# Autodesk Inventor assembly: Carburetor
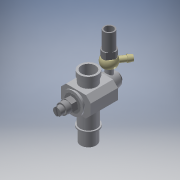
[picture p0: Inventor's stored thumbnail of the model, 180x180]
Saved by Autodesk Inventor 2016 (Build 200138000, 138)
## iProperties
Created: 2012-08-25
Part Number: Carburetor
Document SubType Name: Assembly
Designer: John
Author: John
## Documents named in this file (8)
- C:\File Storage\Autodesk\Inventor 2016 Projects\Ex_Files_Inventor_2016_EssT\Exercise Files\02_Navigating the interface\02_01\Carburetor.iam
- C:\File Storage\Autodesk\Inventor 2016 Projects\Ex_Files_Inventor_2016_EssT\Exercise Files\02_Navigating the interface\02_01\Gas Regulator.ipt
- C:\File Storage\Autodesk\Inventor 2016 Projects\Ex_Files_Inventor_2016_EssT\Exercise Files\02_Navigating the interface\02_01\Mixture Control.ipt
- C:\File Storage\Autodesk\Inventor 2016 Projects\Ex_Files_Inventor_2016_EssT\Exercise Files\02_Navigating the interface\02_01\Air Adjuster.ipt
- C:\File Storage\Autodesk\Inventor 2016 Projects\Ex_Files_Inventor_2016_EssT\Exercise Files\02_Navigating the interface\02_01\Hex Cap.ipt
- C:\File Storage\Autodesk\Inventor 2016 Projects\Ex_Files_Inventor_2016_EssT\Exercise Files\02_Navigating the interface\02_01\Fuel Intake.ipt
- C:\File Storage\Autodesk\Inventor 2016 Projects\Ex_Files_Inventor_2016_EssT\Exercise Files\02_Navigating the interface\02_01\Fuel Adjuster.ipt
- C:\File Storage\Autodesk\Inventor 2016 Projects\Ex_Files_Inventor_2016_EssT\Exercise Files\02_Navigating the interface\02_01\Carburetor Housing_v3.ipt
## Components (7 placed, 7 different names)
1. Carburetor Housing_v3:2 — Mate:6, Mate:7, Mate:10, Flush:1, Flush:2
2. Gas Regulator:1 — Mate:6, Flush:1
3. Mixture Control:1 — Flush:2
4. Air Adjuster:1
5. Hex Cap:1
6. Fuel Intake:1 — Mate:8, Mate:9, Mate:10
7. Fuel Adjuster:1 — Mate:7, Mate:8, Mate:9
## Relationships (12: Mate 10, Flush 2)
- [Mate]: Gas Regulator:1 ↔ Mixture Control:1
- [Mate]: Mixture Control:1 ↔ Air Adjuster:1
- [Mate]: Mixture Control:1 ↔ Hex Cap:1
- [Mate]: Mixture Control:1 ↔ Hex Cap:1
- [Mate] (3.175 mm): Mixture Control:1 ↔ Air Adjuster:1
- Mate:6: Carburetor Housing_v3:2 ↔ Gas Regulator:1
- Mate:7: Carburetor Housing_v3:2 ↔ Fuel Adjuster:1
- Mate:8: Fuel Intake:1 ↔ Fuel Adjuster:1
- Mate:9: Fuel Intake:1 ↔ Fuel Adjuster:1
- Mate:10: Carburetor Housing_v3:2 ↔ Fuel Intake:1
- Flush:1 (-1.27 mm): Carburetor Housing_v3:2 ↔ Gas Regulator:1
- Flush:2: Carburetor Housing_v3:2 ↔ Mixture Control:1
